# Autodesk Inventor assembly: Fume Extractor V1
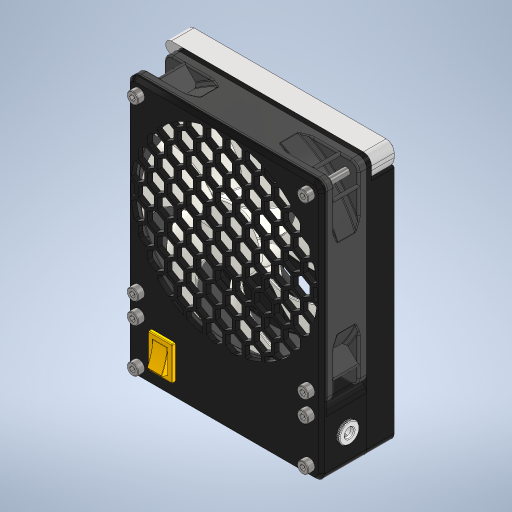
[picture p0: Inventor's stored thumbnail of the model, 512x512]
Saved by Autodesk Inventor 2023.2 (Build 272271000, 271)
## iProperties
Created: 2023-08-15
Part Number: Fume Extractor V1
Document SubType Name: Assembly
Designer: Nathan Cai
Author: Nathan Cai
## Documents named in this file (9)
- E:\Documents\Inventor\Solder Fume Extractor\Fume Extractor V1.iam
- E:\Documents\Inventor\Solder Fume Extractor\120mm Computer Fan v1\120mm Computer Fan v1.ipt
- E:\Documents\Inventor\Solder Fume Extractor\Connector_5,5-2,1_DC00990-B\Connector_5,5-2,1_DC00990-B.ipt
- E:\Documents\Inventor\Solder Fume Extractor\Rocker Switch\Rocker Switch.ipt
- E:\Documents\Inventor\Solder Fume Extractor\Face Plate.ipt
- E:\Documents\Inventor\Solder Fume Extractor\Mid Plate.ipt
- E:\Documents\Inventor\Solder Fume Extractor\Back Plate.ipt
- E:\Documents\Inventor\Solder Fume Extractor\Lid.ipt
- E:\Documents\Inventor\Content Center Files\R2023\en-US\U 2494(1)\Unbrako - M4 x  50(6).ipt
## Components (15 placed, 8 different names)
1. 120mm Computer Fan v1:1 — Mate:2, Mate:3, Mate:4, Mate:5
2. Connector_5,5-2,1_DC00990-B:1 — Mate:2, Mate:9
3. Rocker Switch:1 — Mate:6, Mate:7, Mate:8
4. Face Plate:1 — Mate:3, Mate:4, Mate:5, Mate:6, Mate:7, Mate:8, Mate:9, Mate:10, Flush:1, Flush:2, Flush:3, Flush:4, Mate:15, Mate:16, Mate:17, Mate:18, Mate:19, Mate:20, Mate:21, Mate:22, Mate:23, Mate:24, Mate:25, Mate:26, Mate:27, Mate:28, Mate:29, Mate:30
5. Mid Plate:1 — Mate:10, Flush:1, Flush:2, Mate:11, Mate:12, Mate:13, Mate:14
6. Back Plate:1 — Mate:11, Flush:3, Flush:4
7. Lid:1 — Mate:12, Mate:13, Mate:14
8. Unbrako Hex Socket Cap - Metric M4 x 50:1 — Mate:15, Mate:16
9. Unbrako Hex Socket Cap - Metric M4 x 50:2 — Mate:17, Mate:18
10. Unbrako Hex Socket Cap - Metric M4 x 50:3 — Mate:19, Mate:20
11. Unbrako Hex Socket Cap - Metric M4 x 50:4 — Mate:21, Mate:22
12. Unbrako Hex Socket Cap - Metric M4 x 50:5 — Mate:23, Mate:24
13. Unbrako Hex Socket Cap - Metric M4 x 50:6 — Mate:25, Mate:26
14. Unbrako Hex Socket Cap - Metric M4 x 50:7 — Mate:27, Mate:28
15. Unbrako Hex Socket Cap - Metric M4 x 50:8 — Mate:29, Mate:30
## Relationships (33: Mate 29, Flush 4)
- Mate:2: 120mm Computer Fan v1:1 ↔ Connector_5,5-2,1_DC00990-B:1
- Mate:3: 120mm Computer Fan v1:1 ↔ Face Plate:1
- Mate:4: 120mm Computer Fan v1:1 ↔ Face Plate:1
- Mate:5: 120mm Computer Fan v1:1 ↔ Face Plate:1
- Mate:6: Rocker Switch:1 ↔ Face Plate:1
- Mate:7 (-10 mm): Rocker Switch:1 ↔ Face Plate:1
- Mate:8 (-15 mm): Rocker Switch:1 ↔ Face Plate:1
- Mate:9: Connector_5,5-2,1_DC00990-B:1 ↔ Face Plate:1
- Mate:10: Face Plate:1 ↔ Mid Plate:1
- Flush:1: Face Plate:1 ↔ Mid Plate:1
- Flush:2: Face Plate:1 ↔ Mid Plate:1
- Mate:11: Mid Plate:1 ↔ Back Plate:1
- Flush:3: Face Plate:1 ↔ Back Plate:1
- Flush:4: Face Plate:1 ↔ Back Plate:1
- Mate:12: Mid Plate:1 ↔ Lid:1
- Mate:13: Mid Plate:1 ↔ Lid:1
- Mate:14: Mid Plate:1 ↔ Lid:1
- Mate:15: Face Plate:1 ↔ Unbrako Hex Socket Cap - Metric M4 x 50:1
- Mate:16: Face Plate:1 ↔ Unbrako Hex Socket Cap - Metric M4 x 50:1
- Mate:17: Face Plate:1 ↔ Unbrako Hex Socket Cap - Metric M4 x 50:2
- Mate:18: Face Plate:1 ↔ Unbrako Hex Socket Cap - Metric M4 x 50:2
- Mate:19: Face Plate:1 ↔ Unbrako Hex Socket Cap - Metric M4 x 50:3
- Mate:20: Face Plate:1 ↔ Unbrako Hex Socket Cap - Metric M4 x 50:3
- Mate:21: Face Plate:1 ↔ Unbrako Hex Socket Cap - Metric M4 x 50:4
- Mate:22: Face Plate:1 ↔ Unbrako Hex Socket Cap - Metric M4 x 50:4
- Mate:23: Face Plate:1 ↔ Unbrako Hex Socket Cap - Metric M4 x 50:5
- Mate:24: Face Plate:1 ↔ Unbrako Hex Socket Cap - Metric M4 x 50:5
- Mate:25: Face Plate:1 ↔ Unbrako Hex Socket Cap - Metric M4 x 50:6
- Mate:26: Face Plate:1 ↔ Unbrako Hex Socket Cap - Metric M4 x 50:6
- Mate:27: Face Plate:1 ↔ Unbrako Hex Socket Cap - Metric M4 x 50:7
- Mate:28: Face Plate:1 ↔ Unbrako Hex Socket Cap - Metric M4 x 50:7
- Mate:29: Face Plate:1 ↔ Unbrako Hex Socket Cap - Metric M4 x 50:8
- Mate:30: Face Plate:1 ↔ Unbrako Hex Socket Cap - Metric M4 x 50:8
